# Autodesk Inventor assembly: Ensemble1
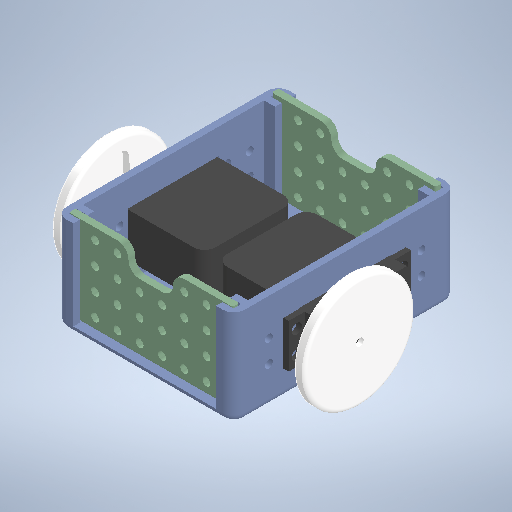
[picture p0: Inventor's stored thumbnail of the model, 512x512]
Saved by Autodesk Inventor 2025 (Build 290162000, 162)
## iProperties
Created: 2024-09-05
Part Number: Ensemble1
Document SubType Name: Assembly
Designer: chass
Author: chass
## Documents named in this file (5)
- C:\Users\chass\Documents\Inventor\Projets\Hackathon\Ensemble1.iam
- C:\Users\chass\Documents\Inventor\Projets\Hackathon\servomoteur_roues.ipt
- C:\Users\chass\Documents\Inventor\Projets\Hackathon\chassis.ipt
- C:\Users\chass\Documents\Inventor\Projets\Hackathon\plaque.ipt
- C:\Users\chass\Documents\Inventor\Projets\Hackathon\roue.ipt
## Components (7 placed, 4 different names)
1. servomoteur_roues:1 — Placage:15, Placage:16
2. servomoteur_roues:2 — Placage:12, Placage:13, Placage:14, Placage:17, Placage:18
3. chassis:1 — Placage:8, Placage:9, Placage:10, Placage:11, Placage:12, Placage:13, Placage:14
4. plaque:1 — Placage:8, Placage:9
5. plaque:2 — Placage:10, Placage:11
6. roue:1 — Placage:15, Placage:16
7. roue:2 — Placage:17, Placage:18
## Relationships (11: Mate 11)
- Placage:8 [Mate]: chassis:1 ↔ plaque:1
- Placage:9 [Mate]: chassis:1 ↔ plaque:1
- Placage:10 [Mate]: chassis:1 ↔ plaque:2
- Placage:11 [Mate]: chassis:1 ↔ plaque:2
- Placage:12 [Mate]: servomoteur_roues:2 ↔ chassis:1
- Placage:13 [Mate]: servomoteur_roues:2 ↔ chassis:1
- Placage:14 [Mate]: servomoteur_roues:2 ↔ chassis:1
- Placage:15 [Mate]: servomoteur_roues:1 ↔ roue:1
- Placage:16 [Mate]: servomoteur_roues:1 ↔ roue:1
- Placage:17 [Mate]: servomoteur_roues:2 ↔ roue:2
- Placage:18 [Mate]: servomoteur_roues:2 ↔ roue:2
